# Autodesk Inventor assembly: Сборка1
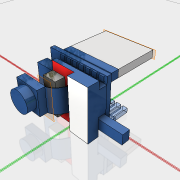
[picture p0: Inventor's stored thumbnail of the model, 180x180]
Saved by Autodesk Inventor 2021.2 (Build 252289000, 289)
## iProperties
Created: 2025-10-22
Part Number: Сборка1
Document SubType Name: Assembly
Designer: Захаров
Author: Захаров
## Documents named in this file (4)
- C:\Users\User\Documents\CaseARHead1\Сборка1.iam
- C:\Users\User\Documents\CaseARHead1\ЛЦМК.00002.00.00.00.00.01.ipt
- C:\Users\User\Documents\CaseARHead1\Сборка2.iam
- C:\Users\User\Documents\CaseARHead1\ЛЦМК.00002.00.00.00.00.21 Контакты.ipt
## Components (4 placed, 3 different names)
1. ЛЦМК.00002.00.00.00.00.01:1
2. Сборка2:1 [sub-assembly] — Совмещение:1, Совмещение:2
3. ЛЦМК.00002.00.00.00.00.01:2 — Совмещение:1, Совмещение:2, Совмещение:3, Заподлицо:1, Заподлицо:2
4. ЛЦМК.00002.00.00.00.00.21 Контакты:1 — Совмещение:3, Заподлицо:1, Заподлицо:2
## Relationships (5: Mate 3, Flush 2)
- Совмещение:1 [Mate]: Сборка2:1 ↔ ЛЦМК.00002.00.00.00.00.01:2
- Совмещение:2 [Mate]: Сборка2:1 ↔ ЛЦМК.00002.00.00.00.00.01:2
- Совмещение:3 [Mate]: ЛЦМК.00002.00.00.00.00.01:2 ↔ ЛЦМК.00002.00.00.00.00.21 Контакты:1
- Заподлицо:1 [Flush]: ЛЦМК.00002.00.00.00.00.01:2 ↔ ЛЦМК.00002.00.00.00.00.21 Контакты:1
- Заподлицо:2 [Flush]: ЛЦМК.00002.00.00.00.00.01:2 ↔ ЛЦМК.00002.00.00.00.00.21 Контакты:1
